# Autodesk Inventor assembly: Amortisseur
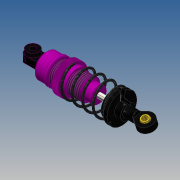
[picture p0: Inventor's stored thumbnail of the model, 180x180]
Saved by Autodesk Inventor 2021.3 (Build 253353000, 353)
## iProperties
Created: 2023-04-12
Part Number: Amortisseur
Document SubType Name: Assembly
Designer: cedric.clivaz
Author: cedric.clivaz
## Documents named in this file (8)
- Y:\cedric.clivaz\Test\Amortisseur\Amortisseur.iam
- Y:\cedric.clivaz\Test\Amortisseur\Corps.ipt
- Y:\cedric.clivaz\Test\Amortisseur\Verin.ipt
- Y:\cedric.clivaz\Test\Amortisseur\Tete_verin.ipt
- Y:\cedric.clivaz\Test\Amortisseur\Boule_tete_verin.ipt
- Y:\cedric.clivaz\Test\Amortisseur\Rondelle.ipt
- Y:\cedric.clivaz\Test\Amortisseur\Ecrou.ipt
- Y:\cedric.clivaz\Test\Amortisseur\Ressort.ipt
## Components (7 placed, 7 different names)
1. Corps:1 — Mate:1, Mate:4, Mate:7, Mate:8, Mate:9
2. Verin:1 — Mate:1, Mate:2, Mate:3
3. Tete_verin:1 — Mate:2, Mate:3, Mate:4, Tangent:1, Mate:5, Mate:6
4. Boule_tete_verin:1 — Tangent:1
5. Rondelle:1 — Mate:5, Mate:6, Mate:11
6. Ecrou:1 — Mate:7, Mate:8, Mate:10
7. Ressort:1 — Mate:9, Mate:10, Mate:11
## Relationships (12: Mate 11, Tangent 1)
- Mate:1: Corps:1 ↔ Verin:1
- Mate:2: Verin:1 ↔ Tete_verin:1
- Mate:3: Verin:1 ↔ Tete_verin:1
- Mate:4 (39.962 mm): Corps:1 ↔ Tete_verin:1
- Tangent:1: Tete_verin:1 ↔ Boule_tete_verin:1
- Mate:5: Tete_verin:1 ↔ Rondelle:1
- Mate:6: Tete_verin:1 ↔ Rondelle:1
- Mate:7: Corps:1 ↔ Ecrou:1
- Mate:8 (3.126 mm): Corps:1 ↔ Ecrou:1
- Mate:9: Corps:1 ↔ Ressort:1
- Mate:10: Ecrou:1 ↔ Ressort:1
- Mate:11: Rondelle:1 ↔ Ressort:1
